# Autodesk Inventor assembly: Segment_Small_Ass
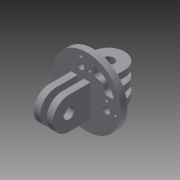
[picture p0: Inventor's stored thumbnail of the model, 180x180]
Saved by Autodesk Inventor 2014 SP1 (Build 180222100, 222)
## iProperties
Created: 2014-03-20
Part Number: Segment_Small_Ass
Document SubType Name: Assembly
Designer: ehagerup
Author: ehagerup
## Documents named in this file (4)
- C:\Users\ehagerup\SkyDrive\Documents\Mechanical Sketches\Animatronic Tail V4\Segment_Small_Ass.iam
- C:\Users\ehagerup\SkyDrive\Documents\Mechanical Sketches\Animatronic Tail V4\Segment_Small.ipt
- C:\Users\ehagerup\SkyDrive\Documents\Mechanical Sketches\Animatronic Tail V4\Connector_3.ipt
- C:\Users\ehagerup\SkyDrive\Documents\Mechanical Sketches\Animatronic Tail V4\Connector_2.ipt
## Components (6 placed, 3 different names)
1. Segment_Small:1 — Flush:7, Mate:1, Mate:2, Mate:3, Flush:8, Mate:4, Mate:5, Mate:6, Mate:7
2. Connector_3:1 — Flush:1, Flush:6, Flush:7, Mate:1, Mate:2
3. Connector_3:2 — Flush:1, Flush:6, Mate:3
4. Connector_2:1 — Flush:3, Flush:4, Mate:7
5. Connector_2:2 — Flush:2, Flush:3, Flush:4, Flush:5, Mate:6
6. Connector_2:3 — Flush:2, Flush:5, Flush:8, Mate:4, Mate:5
## Relationships (15: Flush 8, Mate 7)
- Flush:1: Connector_3:1 ↔ Connector_3:2
- Flush:2: Connector_2:2 ↔ Connector_2:3
- Flush:3: Connector_2:1 ↔ Connector_2:2
- Flush:4: Connector_2:1 ↔ Connector_2:2
- Flush:5: Connector_2:2 ↔ Connector_2:3
- Flush:6: Connector_3:1 ↔ Connector_3:2
- Flush:7: Segment_Small:1 ↔ Connector_3:1
- Mate:1: Segment_Small:1 ↔ Connector_3:1
- Mate:2: Segment_Small:1 ↔ Connector_3:1
- Mate:3: Segment_Small:1 ↔ Connector_3:2
- Flush:8: Segment_Small:1 ↔ Connector_2:3
- Mate:4: Segment_Small:1 ↔ Connector_2:3
- Mate:5: Segment_Small:1 ↔ Connector_2:3
- Mate:6: Segment_Small:1 ↔ Connector_2:2
- Mate:7: Segment_Small:1 ↔ Connector_2:1
